# Autodesk Inventor assembly: Hand
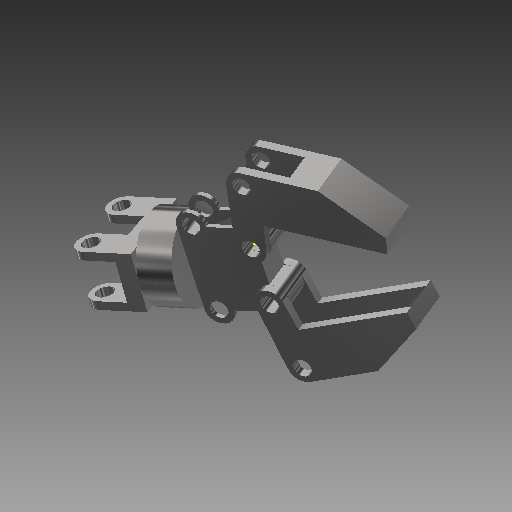
[picture p0: Inventor's stored thumbnail of the model, 512x512]
Saved by Autodesk Inventor 2019 (Build 230136000, 136)
## iProperties
Created: 2018-12-28
Part Number: Hand
Material: 常规
Document SubType Name: Assembly
Designer: JianQiao Hu
Author: JianQiao Hu
## Documents named in this file (4)
- C:\Users\Administrator\Desktop\机械产品数字化设计大赛\月球机器人\机械臂\DruggerArm\Hand.iam
- C:\Users\Administrator\Desktop\机械产品数字化设计大赛\月球机器人\机械臂\DruggerArm\Wrist.ipt
- C:\Users\Administrator\Desktop\机械产品数字化设计大赛\月球机器人\机械臂\DruggerArm\Pam.ipt
- C:\Users\Administrator\Desktop\机械产品数字化设计大赛\月球机器人\机械臂\DruggerArm\Finger.ipt
## Components (4 placed, 3 different names)
1. Wrist:1 — 配合:1, 配合:2
2. Pam:1 — 配合:1, 配合:2, 配合:3, 配合:4, 配合:5, 配合:6
3. Finger:1 — 配合:4, 配合:5, 转动:1
4. Finger:2 — 配合:3, 配合:6, 转动:1
## Relationships (7: Mate 6, RelateRotation 1)
- 配合:1 [Mate]: Wrist:1 ↔ Pam:1
- 配合:2 [Mate]: Wrist:1 ↔ Pam:1
- 配合:3 [Mate]: Pam:1 ↔ Finger:2
- 配合:4 [Mate]: Pam:1 ↔ Finger:1
- 配合:5 [Mate]: Pam:1 ↔ Finger:1
- 配合:6 [Mate]: Pam:1 ↔ Finger:2
- 转动:1 [RelateRotation] (1 ul): Finger:1 ↔ Finger:2
